# Autodesk Inventor assembly: hooks and faceplate
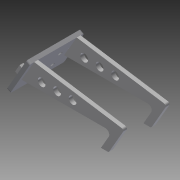
[picture p0: Inventor's stored thumbnail of the model, 180x180]
Saved by Autodesk Inventor 2013 (Build 170138000, 138)
## iProperties
Created: 2013-02-10
Part Number: hooks and faceplate
Document SubType Name: Assembly
Designer: Arpan
Author: Arpan
## Documents named in this file (3)
- C:\Users\Arpan\Documents\GitHub\frc2013CAD\hooks and faceplate.iam
- C:\Users\Arpan\Documents\GitHub\frc2013CAD\Cimber actual\hook.ipt
- C:\Users\Arpan\Documents\GitHub\frc2013CAD\Cimber actual\hook faceplate.ipt
## Components (3 placed, 2 different names)
1. hook:1 — Mate:3, Mate:4, Flush:1
2. hook:2 — Mate:1, Mate:2, Flush:1, Mate:5
3. hook faceplate:1 — Mate:1, Mate:2, Mate:3, Mate:4, Mate:5
## Relationships (6: Mate 5, Flush 1)
- Mate:1: hook:2 ↔ hook faceplate:1
- Mate:2: hook:2 ↔ hook faceplate:1
- Mate:3: hook:1 ↔ hook faceplate:1
- Mate:4: hook:1 ↔ hook faceplate:1
- Flush:1: hook:1 ↔ hook:2
- Mate:5: hook:2 ↔ hook faceplate:1
